# Autodesk Inventor assembly: Robot_base
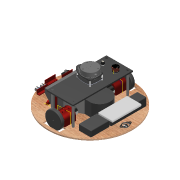
[picture p0: Inventor's stored thumbnail of the model, 180x180]
Saved by Autodesk Inventor 2020 (Build 240168000, 168)
## iProperties
Created: 2022-08-27
Part Number: Robot_base
Document SubType Name: Assembly
Designer: Umair
Author: Umair
## Documents named in this file (24)
- C:\Users\pc\Dropbox\Umair\SCHOOL\1 Ma\Masterthesis\CAD\Robot_base.iam
- C:\Users\pc\Dropbox\Umair\SCHOOL\1 Ma\Masterthesis\CAD\Robot_base.ipt
- C:\Users\pc\Dropbox\Umair\SCHOOL\1 Ma\Masterthesis\CAD\37D mm Metal Gearbox Polulu.ipt
- C:\Users\pc\Dropbox\Umair\SCHOOL\1 Ma\Masterthesis\CAD\bull_eye_wheel.ipt
- C:\Users\pc\Dropbox\Umair\SCHOOL\1 Ma\Masterthesis\CAD\Wheels.ipt
- C:\Users\pc\Dropbox\Umair\SCHOOL\1 Ma\Masterthesis\CAD\vacuum_piece_1.ipt
- C:\Users\pc\Dropbox\Umair\SCHOOL\1 Ma\Masterthesis\CAD\vacuum_endpiece.ipt
- C:\Users\pc\Dropbox\Umair\SCHOOL\1 Ma\Masterthesis\CAD\vacuum_bin_holder.ipt
- C:\Users\pc\Dropbox\Umair\SCHOOL\1 Ma\Masterthesis\CAD\Motor_mount_Left.ipt
- C:\Users\pc\Dropbox\Umair\SCHOOL\1 Ma\Masterthesis\CAD\Sharp_IR_holder.ipt
- C:\Users\pc\Dropbox\Umair\SCHOOL\1 Ma\Masterthesis\CAD\platform_plate.ipt
- C:\Users\pc\Dropbox\Umair\SCHOOL\1 Ma\Masterthesis\CAD\IR_holder.ipt
- C:\Users\pc\Dropbox\Umair\SCHOOL\1 Ma\Masterthesis\CAD\platform_holder.ipt
- C:\Users\pc\Dropbox\Umair\SCHOOL\1 Ma\Masterthesis\CAD\Piece2.ipt
- C:\Users\pc\Dropbox\Umair\SCHOOL\1 Ma\Masterthesis\CAD\piece3.ipt
- C:\Users\pc\Dropbox\Umair\SCHOOL\1 Ma\Masterthesis\CAD\piece1.ipt
- C:\Users\pc\Dropbox\Umair\SCHOOL\1 Ma\Masterthesis\CAD\LIPO.ipt
- C:\Users\pc\Dropbox\Umair\SCHOOL\1 Ma\Masterthesis\CAD\Powerbank.ipt
- C:\Users\pc\Dropbox\Umair\SCHOOL\1 Ma\Masterthesis\CAD\RBPI.ipt
- C:\Users\pc\Dropbox\Umair\SCHOOL\1 Ma\Masterthesis\CAD\RP-lidar-A1\RP-lidar-A1.iam
- C:\Users\pc\Dropbox\Umair\SCHOOL\1 Ma\Masterthesis\CAD\SharpIRsensor.ipt
- C:\Users\pc\Dropbox\Umair\SCHOOL\1 Ma\Masterthesis\CAD\HC-SR04.ipt
- C:\Users\pc\Dropbox\Umair\SCHOOL\1 Ma\Masterthesis\CAD\Fuse holder.ipt
- C:\Users\pc\Dropbox\Umair\SCHOOL\1 Ma\Masterthesis\CAD\E-Stop.ipt
## Components (31 placed, 23 different names)
1. Robot_base:1 — Mate:1, Mate:2, Flush:1, Mate:3, Mate:4, Mate:5, Mate:6, Mate:11, Mate:12, Mate:14, Mate:15, Flush:4, Mate:17, Mate:18, Mate:20, Mate:21, Mate:22, Mate:23, Flush:7, Flush:8, Flush:9, Flush:10, Mate:26, Mate:27, Mate:28, Mate:29, Mate:30, Mate:41, Mate:43, Mate:45, Mate:49
2. 37D mm Metal Gearbox Polulu:1 — Mate:7, Mate:9, Mate:16, Flush:3
3. bull_eye_wheel:1 — Mate:3, Mate:4
4. 37D mm Metal Gearbox Polulu:2 — Mate:8, Mate:10, Mate:13, Flush:2
5. Wheels:1 — Mate:16, Flush:3
6. Wheels:2 — Mate:13, Flush:2
7. vacuum_piece_1:1 — Flush:4, Mate:17, Mate:18, Mate:19, Flush:5, Flush:6
8. vacuum_endpiece:1 — Mate:19, Flush:5, Flush:6
9. vacuum_bin_holder:1 — Mate:29, Mate:31, Flush:12, Mate:42
10. vacuum_bin_holder:2 — Mate:30, Mate:32, Flush:12
11. Motor_mount_Left:1 — Mate:5, Mate:7, Mate:9, Mate:14, Mate:15
12. Motor_mount_Left:2 — Mate:6, Mate:8, Mate:10, Mate:11, Mate:12
13. Sharp_IR_holder:1 — Mate:27, Flush:13, Mate:50
14. platform_plate:1 — Flush:15, Mate:33, Mate:34, Mate:46, Mate:47, Mate:51, Flush:17, Flush:18, Mate:52
15. IR_holder:1 — Mate:28, Flush:13, Flush:14, Mate:48, Flush:16
16. platform_holder:1 — Mate:20, Flush:7, Mate:34
17. platform_holder:2 — Mate:21, Flush:9
18. platform_holder:3 — Mate:23, Flush:10
19. platform_holder:4 — Mate:22, Flush:8, Flush:15, Mate:33
20. Sharp_IR_holder:2 — Mate:26, Flush:14
21. Piece2:1 — Mate:35, Mate:36, Mate:37, Mate:40
22. piece3:1 — Mate:36, Mate:37, Mate:38, Mate:39, Mate:40
23. piece1:1 — Mate:35, Mate:38, Mate:39, Mate:41, Mate:42
24. LIPO:1 — Mate:43, Mate:44
25. Powerbank:1 — Mate:44
26. RBPI:1 — Mate:45
27. RP-lidar-A1:1 [sub-assembly] — Mate:46, Mate:47
28. SharpIRsensor:1 — Mate:50
29. HC-SR04:1 — Mate:48, Mate:49, Flush:16
30. Fuse holder:1 — Flush:18, Mate:52
31. E-Stop:1 — Mate:51, Flush:17
## Relationships (67: Mate 50, Flush 17)
- Mate:1: Robot_base:1
- Mate:2: Robot_base:1
- Flush:1: Robot_base:1
- Mate:3 (-10 mm): Robot_base:1 ↔ bull_eye_wheel:1
- Mate:4: Robot_base:1 ↔ bull_eye_wheel:1
- Mate:5: Robot_base:1 ↔ Motor_mount_Left:1
- Mate:6: Robot_base:1 ↔ Motor_mount_Left:2
- Mate:7: 37D mm Metal Gearbox Polulu:1 ↔ Motor_mount_Left:1
- Mate:8 (9 mm): 37D mm Metal Gearbox Polulu:2 ↔ Motor_mount_Left:2
- Mate:9 (8.5 mm): 37D mm Metal Gearbox Polulu:1 ↔ Motor_mount_Left:1
- Mate:10: 37D mm Metal Gearbox Polulu:2 ↔ Motor_mount_Left:2
- Mate:11: Robot_base:1 ↔ Motor_mount_Left:2
- Mate:12: Robot_base:1 ↔ Motor_mount_Left:2
- Mate:13: 37D mm Metal Gearbox Polulu:2 ↔ Wheels:2
- Flush:2 (-5 mm): 37D mm Metal Gearbox Polulu:2 ↔ Wheels:2
- Mate:14: Robot_base:1 ↔ Motor_mount_Left:1
- Mate:15: Robot_base:1 ↔ Motor_mount_Left:1
- Mate:16: 37D mm Metal Gearbox Polulu:1 ↔ Wheels:1
- Flush:3 (-5 mm): 37D mm Metal Gearbox Polulu:1 ↔ Wheels:1
- Flush:4 (-1 mm): Robot_base:1 ↔ vacuum_piece_1:1
- Mate:17 (1 mm): Robot_base:1 ↔ vacuum_piece_1:1
- Mate:18 (1 mm): Robot_base:1 ↔ vacuum_piece_1:1
- Mate:19: vacuum_piece_1:1 ↔ vacuum_endpiece:1
- Flush:5: vacuum_piece_1:1 ↔ vacuum_endpiece:1
- Flush:6: vacuum_piece_1:1 ↔ vacuum_endpiece:1
- Mate:20: Robot_base:1 ↔ platform_holder:1
- Mate:21: Robot_base:1 ↔ platform_holder:2
- Mate:22: Robot_base:1 ↔ platform_holder:4
- Mate:23: Robot_base:1 ↔ platform_holder:3
- Flush:7: Robot_base:1 ↔ platform_holder:1
- Flush:8: Robot_base:1 ↔ platform_holder:4
- Flush:9: Robot_base:1 ↔ platform_holder:2
- Flush:10: Robot_base:1 ↔ platform_holder:3
- Mate:26: Robot_base:1 ↔ Sharp_IR_holder:2
- Mate:27: Robot_base:1 ↔ Sharp_IR_holder:1
- Mate:28: Robot_base:1 ↔ IR_holder:1
- Mate:29: Robot_base:1 ↔ vacuum_bin_holder:1
- Mate:30: Robot_base:1 ↔ vacuum_bin_holder:2
- Mate:31 (-100 mm): vacuum_bin_holder:1
- Mate:32 (100 mm): vacuum_bin_holder:2
- Flush:12: vacuum_bin_holder:1 ↔ vacuum_bin_holder:2
- Flush:13: Sharp_IR_holder:1 ↔ IR_holder:1
- Flush:14 (20 mm): IR_holder:1 ↔ Sharp_IR_holder:2
- Flush:15: platform_plate:1 ↔ platform_holder:4
- Mate:33: platform_plate:1 ↔ platform_holder:4
- Mate:34: platform_plate:1 ↔ platform_holder:1
- Mate:35: Piece2:1 ↔ piece1:1
- Mate:36: Piece2:1 ↔ piece3:1
- Mate:37: Piece2:1 ↔ piece3:1
- Mate:38: piece3:1 ↔ piece1:1
- Mate:39 (62 mm): piece3:1 ↔ piece1:1
- Mate:40 (62 mm): Piece2:1 ↔ piece3:1
- Mate:41: Robot_base:1 ↔ piece1:1
- Mate:42: vacuum_bin_holder:1 ↔ piece1:1
- Mate:43: Robot_base:1 ↔ LIPO:1
- Mate:44: LIPO:1 ↔ Powerbank:1
- Mate:45: Robot_base:1 ↔ RBPI:1
- Mate:46: platform_plate:1 ↔ RP-lidar-A1:1
- Mate:47: platform_plate:1 ↔ RP-lidar-A1:1
- Mate:48: IR_holder:1 ↔ HC-SR04:1
- Mate:49: Robot_base:1 ↔ HC-SR04:1
- Flush:16 (2.5 mm): IR_holder:1 ↔ HC-SR04:1
- Mate:50: Sharp_IR_holder:1 ↔ SharpIRsensor:1
- Mate:51: platform_plate:1 ↔ E-Stop:1
- Flush:17 (-22 mm): platform_plate:1 ↔ E-Stop:1
- Flush:18 (-12 mm): platform_plate:1 ↔ Fuse holder:1
- Mate:52: platform_plate:1 ↔ Fuse holder:1
